# Autodesk Inventor assembly: Pancake_Tilted Tube Assy_3 Lanes
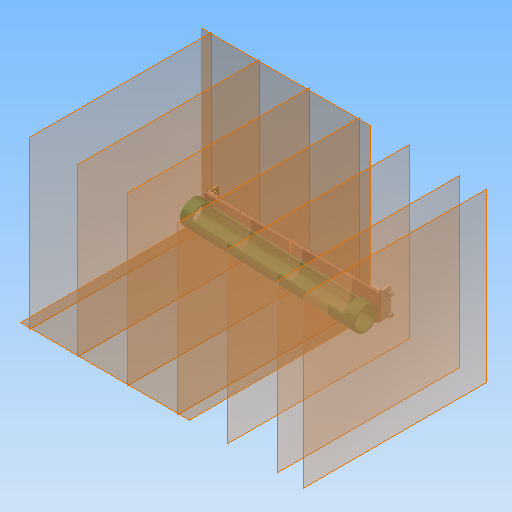
[picture p0: Inventor's stored thumbnail of the model, 512x512]
Saved by Autodesk Inventor 2018.1 (Build 221171000, 171)
## iProperties
Created: 2019-02-21
Part Number: Pancake_Tilted Tube Assy_3 Lanes
Document SubType Name: Assembly
Designer: James
Author: James
## Documents named in this file (8)
- C:\Users\admin\Desktop\Ball-Machine\Pancake Sort\Pancake - 3 Lanes\Pancake_Tilted Tube Assy_3 Lanes.iam
- C:\Users\admin\Desktop\Ball-Machine\Prototype CAD\Selection Sort - 40mm\Nyloc Nut - M4.ipt
- C:\Users\admin\Desktop\Ball-Machine\Pancake Sort\Pancake_Angle Bracket.ipt
- C:\Users\admin\Desktop\Ball-Machine\Prototype CAD\Selection Sort - 40mm\Socket Csk Screw - (A2) - M4 x  12.ipt
- C:\Users\admin\Desktop\Ball-Machine\Prototype CAD\Selection Sort - 40mm\Socket Csk Screw - (A2) - M4 x  16.ipt
- C:\Users\admin\Desktop\Ball-Machine\Prototype CAD\Selection Sort - 40mm\Socket Cap Screw - Standard - (A2) - M4 x 16.ipt
- C:\Users\admin\Desktop\Ball-Machine\Pancake Sort\Pancake - 3 Lanes\Pancake_Tilt Pipe_3 Lanes.ipt
- C:\Users\admin\Desktop\Ball-Machine\Pancake Sort\Pancake - 3 Lanes\Pancake_Tilted Tube Backboard_3 Lanes.ipt
## Components (26 placed, 7 different names)
1. Pancake_Tilted Tube Backboard_3 Lanes:1 — Flush:1, Flush:2, Flush:3, Mate:9, Flush:6, Mate:10, Mate:11, Mate:12, Mate:13, Mate:14, Flush:7, Mate:15, Mate:16, Tangent:1, Tangent:2, Mate:21, Mate:22, Tangent:3, Tangent:4, Tangent:5, Mate:28, Mate:29, Mate:30, Flush:8, Mate:36, Mate:34, Mate:35
2. Pancake_Tilt Pipe_3 Lanes:1 — Tangent:5, Mate:28, Mate:29, Mate:30, Mate:31, Mate:32, Mate:33
3. Pancake_Angle Bracket:1 — Mate:9, Flush:6, Mate:10, Mate:11, Mate:17, Mate:18, Mate:44, Mate:45, Mate:46, Mate:47
4. Pancake_Angle Bracket:2 — Mate:12, Mate:13, Mate:14, Flush:7, Mate:23, Mate:24, Mate:48, Mate:49, Mate:50, Mate:51
5. Nyloc Nut - M4:1 — Mate:18, Mate:20
6. Socket Csk Screw - (A2) - M4 x  12:1 — Mate:15, Tangent:1, Mate:19
7. Nyloc Nut - M4:2 — Mate:17, Mate:19
8. Socket Csk Screw - (A2) - M4 x  12:2 — Mate:16, Tangent:2, Mate:20
9. Nyloc Nut - M4:3 — Mate:23, Mate:26
10. Socket Csk Screw - (A2) - M4 x  12:3 — Mate:21, Tangent:3, Mate:26
11. Nyloc Nut - M4:4 — Mate:24, Mate:25
12. Socket Csk Screw - (A2) - M4 x  12:4 — Mate:22, Tangent:4, Mate:25
13. Nyloc Nut - M4:5 — Mate:36, Mate:38
14. Socket Csk Screw - (A2) - M4 x  16:3 — Mate:31, Flush:10, Mate:39
15. Nyloc Nut - M4:6 — Mate:34, Mate:39
16. Socket Csk Screw - (A2) - M4 x  16:2 — Mate:32, Flush:9, Flush:10, Mate:38
17. Nyloc Nut - M4:7 — Mate:35, Mate:37
18. Socket Csk Screw - (A2) - M4 x  16:1 — Mate:33, Flush:8, Flush:9, Mate:37
19. Nyloc Nut - M4:8 — Flush:12, Mate:47
20. Socket Cap Screw - Standard - (A2) - M4 x 16:1 — Flush:11, Mate:44, Mate:46
21. Nyloc Nut - M4:9 — Flush:12
22. Socket Cap Screw - Standard - (A2) - M4 x 16:2 — Flush:11, Mate:45
23. Nyloc Nut - M4:10 — Flush:14
24. Socket Cap Screw - Standard - (A2) - M4 x 16:3 — Flush:13, Mate:48, Mate:49
25. Nyloc Nut - M4:11 — Flush:14, Mate:51
26. Socket Cap Screw - Standard - (A2) - M4 x 16:4 — Flush:13, Mate:50
## Relationships (59: Mate 42, Flush 12, Tangent 5)
- Flush:1: Pancake_Tilted Tube Backboard_3 Lanes:1
- Flush:2: Pancake_Tilted Tube Backboard_3 Lanes:1
- Flush:3: Pancake_Tilted Tube Backboard_3 Lanes:1
- Mate:9: Pancake_Tilted Tube Backboard_3 Lanes:1 ↔ Pancake_Angle Bracket:1
- Flush:6: Pancake_Tilted Tube Backboard_3 Lanes:1 ↔ Pancake_Angle Bracket:1
- Mate:10: Pancake_Tilted Tube Backboard_3 Lanes:1 ↔ Pancake_Angle Bracket:1
- Mate:11: Pancake_Tilted Tube Backboard_3 Lanes:1 ↔ Pancake_Angle Bracket:1
- Mate:12: Pancake_Tilted Tube Backboard_3 Lanes:1 ↔ Pancake_Angle Bracket:2
- Mate:13: Pancake_Tilted Tube Backboard_3 Lanes:1 ↔ Pancake_Angle Bracket:2
- Mate:14: Pancake_Tilted Tube Backboard_3 Lanes:1 ↔ Pancake_Angle Bracket:2
- Flush:7: Pancake_Tilted Tube Backboard_3 Lanes:1 ↔ Pancake_Angle Bracket:2
- Mate:15: Pancake_Tilted Tube Backboard_3 Lanes:1 ↔ Socket Csk Screw - (A2) - M4 x  12:1
- Mate:16: Pancake_Tilted Tube Backboard_3 Lanes:1 ↔ Socket Csk Screw - (A2) - M4 x  12:2
- Tangent:1: Pancake_Tilted Tube Backboard_3 Lanes:1 ↔ Socket Csk Screw - (A2) - M4 x  12:1
- Tangent:2: Pancake_Tilted Tube Backboard_3 Lanes:1 ↔ Socket Csk Screw - (A2) - M4 x  12:2
- Mate:17: Pancake_Angle Bracket:1 ↔ Nyloc Nut - M4:2
- Mate:18: Pancake_Angle Bracket:1 ↔ Nyloc Nut - M4:1
- Mate:19: Socket Csk Screw - (A2) - M4 x  12:1 ↔ Nyloc Nut - M4:2
- Mate:20: Nyloc Nut - M4:1 ↔ Socket Csk Screw - (A2) - M4 x  12:2
- Mate:21: Pancake_Tilted Tube Backboard_3 Lanes:1 ↔ Socket Csk Screw - (A2) - M4 x  12:3
- Mate:22: Pancake_Tilted Tube Backboard_3 Lanes:1 ↔ Socket Csk Screw - (A2) - M4 x  12:4
- Tangent:3: Pancake_Tilted Tube Backboard_3 Lanes:1 ↔ Socket Csk Screw - (A2) - M4 x  12:3
- Tangent:4: Pancake_Tilted Tube Backboard_3 Lanes:1 ↔ Socket Csk Screw - (A2) - M4 x  12:4
- Mate:23: Pancake_Angle Bracket:2 ↔ Nyloc Nut - M4:3
- Mate:24: Pancake_Angle Bracket:2 ↔ Nyloc Nut - M4:4
- Mate:25: Nyloc Nut - M4:4 ↔ Socket Csk Screw - (A2) - M4 x  12:4
- Mate:26: Nyloc Nut - M4:3 ↔ Socket Csk Screw - (A2) - M4 x  12:3
- Tangent:5: Pancake_Tilted Tube Backboard_3 Lanes:1 ↔ Pancake_Tilt Pipe_3 Lanes:1
- Mate:28: Pancake_Tilted Tube Backboard_3 Lanes:1 ↔ Pancake_Tilt Pipe_3 Lanes:1
- Mate:29: Pancake_Tilted Tube Backboard_3 Lanes:1 ↔ Pancake_Tilt Pipe_3 Lanes:1
- Mate:30: Pancake_Tilted Tube Backboard_3 Lanes:1 ↔ Pancake_Tilt Pipe_3 Lanes:1
- Mate:31: Pancake_Tilt Pipe_3 Lanes:1 ↔ Socket Csk Screw - (A2) - M4 x  16:3
- Mate:32: Pancake_Tilt Pipe_3 Lanes:1 ↔ Socket Csk Screw - (A2) - M4 x  16:2
- Mate:33: Pancake_Tilt Pipe_3 Lanes:1 ↔ Socket Csk Screw - (A2) - M4 x  16:1
- Flush:8 (-5 mm): Pancake_Tilted Tube Backboard_3 Lanes:1 ↔ Socket Csk Screw - (A2) - M4 x  16:1
- Flush:9: Socket Csk Screw - (A2) - M4 x  16:2 ↔ Socket Csk Screw - (A2) - M4 x  16:1
- Flush:10: Socket Csk Screw - (A2) - M4 x  16:3 ↔ Socket Csk Screw - (A2) - M4 x  16:2
- Mate:36: Pancake_Tilted Tube Backboard_3 Lanes:1 ↔ Nyloc Nut - M4:5
- Mate:34: Pancake_Tilted Tube Backboard_3 Lanes:1 ↔ Nyloc Nut - M4:6
- Mate:35: Pancake_Tilted Tube Backboard_3 Lanes:1 ↔ Nyloc Nut - M4:7
- Mate:37: Nyloc Nut - M4:7 ↔ Socket Csk Screw - (A2) - M4 x  16:1
- Mate:38: Nyloc Nut - M4:5 ↔ Socket Csk Screw - (A2) - M4 x  16:2
- Mate:39: Socket Csk Screw - (A2) - M4 x  16:3 ↔ Nyloc Nut - M4:6
- [Mate]: Nyloc Nut - M4:8 ↔ Socket Cap Screw - Standard - (A2) - M4 x 16:1
- [Mate]: Nyloc Nut - M4:9 ↔ Socket Cap Screw - Standard - (A2) - M4 x 16:2
- [Mate]: Nyloc Nut - M4:10 ↔ Socket Cap Screw - Standard - (A2) - M4 x 16:3
- [Mate]: Nyloc Nut - M4:11 ↔ Socket Cap Screw - Standard - (A2) - M4 x 16:4
- Flush:11: Socket Cap Screw - Standard - (A2) - M4 x 16:1 ↔ Socket Cap Screw - Standard - (A2) - M4 x 16:2
- Flush:12: Nyloc Nut - M4:8 ↔ Nyloc Nut - M4:9
- Mate:44 (5 mm): Pancake_Angle Bracket:1 ↔ Socket Cap Screw - Standard - (A2) - M4 x 16:1
- Mate:45: Pancake_Angle Bracket:1 ↔ Socket Cap Screw - Standard - (A2) - M4 x 16:2
- Mate:46: Pancake_Angle Bracket:1 ↔ Socket Cap Screw - Standard - (A2) - M4 x 16:1
- Mate:47: Pancake_Angle Bracket:1 ↔ Nyloc Nut - M4:8
- Flush:13: Socket Cap Screw - Standard - (A2) - M4 x 16:3 ↔ Socket Cap Screw - Standard - (A2) - M4 x 16:4
- Flush:14: Nyloc Nut - M4:10 ↔ Nyloc Nut - M4:11
- Mate:48 (5 mm): Pancake_Angle Bracket:2 ↔ Socket Cap Screw - Standard - (A2) - M4 x 16:3
- Mate:49: Pancake_Angle Bracket:2 ↔ Socket Cap Screw - Standard - (A2) - M4 x 16:3
- Mate:50: Pancake_Angle Bracket:2 ↔ Socket Cap Screw - Standard - (A2) - M4 x 16:4
- Mate:51: Pancake_Angle Bracket:2 ↔ Nyloc Nut - M4:11
## Named parameters: d97_d75_d46 = 0 mm, d81_d97_d75_d46 = 0 mm, d82_d97_d75_d46 = 0 mm, d83_d97_d75_d46 = 0 mm
